# Autodesk Inventor assembly: Powell_1XYAssembly
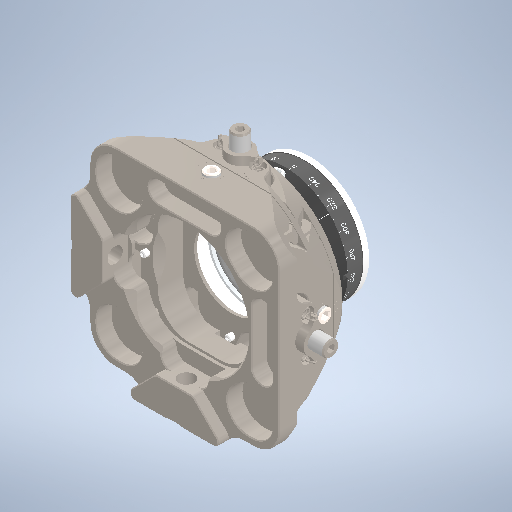
[picture p0: Inventor's stored thumbnail of the model, 512x512]
Saved by Autodesk Inventor 2025.2 (Build 292293000, 293)
## iProperties
Created: 2025-10-16
Part Number: Powell_1XYAssembly
Document SubType Name: Assembly
Designer: monolithic
Author: monolithic
## Documents named in this file (4)
- C:\Users\monolithic\Documents\GitHub\CAD\Monolith\John\Altair_PowellBaseplate_SPIM_ASLM_CTASLM\Assembly\SubAssemblies\Powell_1XYAssembly.iam
- C:\Users\monolithic\Documents\GitHub\CAD\Monolith\John\Altair_PowellBaseplate_SPIM_ASLM_CTASLM\Assembly\SubAssemblies\LRM1-Step.ipt
- C:\Users\monolithic\Documents\GitHub\CAD\Monolith\John\Altair_PowellBaseplate_SPIM_ASLM_CTASLM\Assembly\SubAssemblies\POLARIS-1XY.ipt
- C:\Users\monolithic\Documents\GitHub\CAD\components\ThorLabs\AD9F.ipt
## Components (3 placed, 3 different names)
1. LRM1-Step:1 — Mate:1, Mate:2, Mate:3, Mate:4
2. POLARIS-1XY:1 — Mate:3, Mate:4
3. AD9F:1 — Mate:1, Mate:2
## Relationships (4: Mate 4)
- Mate:1: LRM1-Step:1 ↔ AD9F:1
- Mate:2: LRM1-Step:1 ↔ AD9F:1
- Mate:3: LRM1-Step:1 ↔ POLARIS-1XY:1
- Mate:4: LRM1-Step:1 ↔ POLARIS-1XY:1
